# Autodesk Inventor assembly: ArmSolenoid
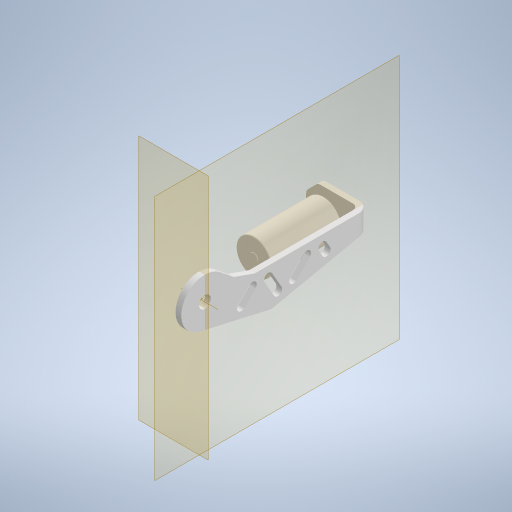
[picture p0: Inventor's stored thumbnail of the model, 512x512]
Saved by Autodesk Inventor 2023 (Build 270158000, 158)
## iProperties
Created: 2023-03-29
Part Number: ArmSolenoid
Document SubType Name: Assembly
Designer: LattePanda
Author: LattePanda
## Documents named in this file (3)
- C:\Users\LattePanda\Desktop\str1ker\parts\external\ArmSolenoid.iam
- C:\Users\LattePanda\Desktop\str1ker\parts\external\ArmSolenoidBody.ipt
- C:\Users\LattePanda\Desktop\str1ker\parts\SolenoidBracket.ipt
## Components (2 placed, 2 different names)
1. ArmSolenoid:1 — Mate:4, Mate:9, Angle:1
2. SolenoidBracket:1 — Mate:4, Mate:7, Mate:8, Mate:9
## Relationships (5: Mate 4, Angle 1)
- Mate:4: ArmSolenoid:1 ↔ SolenoidBracket:1
- Mate:7: SolenoidBracket:1
- Mate:8: SolenoidBracket:1
- Mate:9: ArmSolenoid:1 ↔ SolenoidBracket:1
- Angle:1 (0 deg): ArmSolenoid:1
